# Autodesk Inventor assembly: screwNut
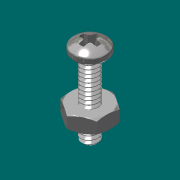
[picture p0: Inventor's stored thumbnail of the model, 180x180]
Saved by Autodesk Inventor 2016 (Build 200138000, 138)
## iProperties
Created: 2016-08-27
Part Number: screwNut
Document SubType Name: Assembly
Designer: sawaiz
Author: sawaiz
## Documents named in this file (3)
- C:\Users\sawaiz\oneDrive\projects\splitFlapDisplay\frame\screwNut.iam
- C:\Users\sawaiz\oneDrive\projects\splitFlapDisplay\frame\4-40Nut.ipt
- C:\Users\sawaiz\oneDrive\projects\splitFlapDisplay\frame\4-40x0.5inPan.ipt
## Components (2 placed, 2 different names)
1. 4-40Nut:1 — Mate:1
2. 4-40x0.5inPan:1 — Mate:1
## Relationships (1: Mate 1)
- Mate:1: 4-40Nut:1 ↔ 4-40x0.5inPan:1
